# Autodesk Inventor assembly: SAR330  x 5 + front couplers
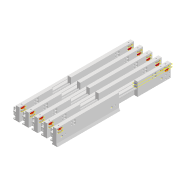
[picture p0: Inventor's stored thumbnail of the model, 180x180]
Saved by Autodesk Inventor 2020 (Build 240168000, 168)
## iProperties
Created: 2019-11-17
Part Number: SAR330  x 5 + front couplers
Document SubType Name: Assembly
Designer: ball
Author: ball
## Documents named in this file (3)
- C:\FTC\FTC8863CAD\2019 Robot\Delivery\SAR330  x 5 + front couplers.iam
- C:\FTC\FTC8863CAD\2019 Robot\Delivery\SAR330 x 4 + regular couplers offset.iam
- C:\FTC\FTC8863CAD\2019 Robot\Delivery\SAR330 + fixed couplers front.iam
## Components (2 placed, 2 different names)
1. SAR330 x 4 + regular couplers offset:1 [sub-assembly] — Mate:1, Mate:2, Mate:3
2. SAR330 + fixed couplers front:1 [sub-assembly] — Mate:1, Mate:2, Mate:3
## Relationships (3: Mate 3)
- Mate:1: SAR330 x 4 + regular couplers offset:1 ↔ SAR330 + fixed couplers front:1
- Mate:2: SAR330 x 4 + regular couplers offset:1 ↔ SAR330 + fixed couplers front:1
- Mate:3: SAR330 x 4 + regular couplers offset:1 ↔ SAR330 + fixed couplers front:1
